# Autodesk Inventor assembly: legg_assembly
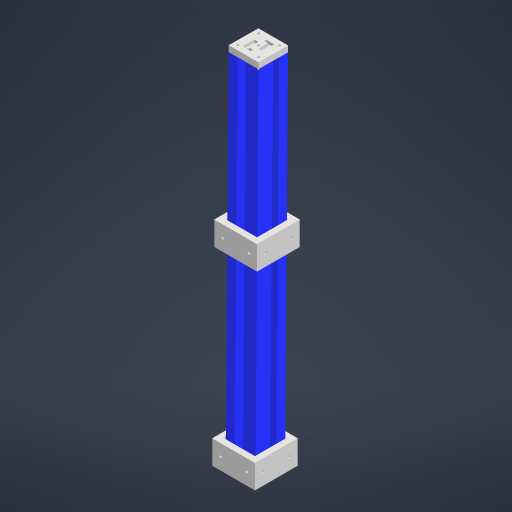
[picture p0: Inventor's stored thumbnail of the model, 512x512]
Saved by Autodesk Inventor 2024 (Build 280153000, 153)
## iProperties
Created: 2023-05-23
Part Number: legg_assembly
Document SubType Name: Assembly
Designer: aasmu
Author: aasmu
## Documents named in this file (4)
- C:\Users\aasmu\Documents\standing_desk\legg_assembly.iam
- C:\Users\aasmu\Documents\standing_desk\1_inner_leg.ipt
- C:\Users\aasmu\Documents\standing_desk\2_inner_leg_top_plate.ipt
- C:\Users\aasmu\Documents\standing_desk\inner_glide_cartrige_full_assembly.iam
## Components (4 placed, 3 different names)
1. 1_inner_leg:1 — Rigid:1, Tangent:1, Tangent:2, Rotation/Translation:1, Tangent:3
2. inner_glide_cartrige_full_assembly:1 [sub-assembly] — Rotation/Translation:1, Tangent:3
3. inner_glide_cartrige_full_assembly:2 [sub-assembly] — Tangent:1, Tangent:2
4. 2_inner_leg_top_plate:1 — Rigid:1
## Relationships (5: Tangent 3, WeldJoint 1, RelateRotateTranslate 1)
- Rigid:1 [WeldJoint]: 1_inner_leg:1 ↔ 2_inner_leg_top_plate:1
- Tangent:1: 1_inner_leg:1 ↔ inner_glide_cartrige_full_assembly:2
- Tangent:2: 1_inner_leg:1 ↔ inner_glide_cartrige_full_assembly:2
- Rotation/Translation:1 [RelateRotateTranslate] (1 mm): 1_inner_leg:1 ↔ inner_glide_cartrige_full_assembly:1
- Tangent:3: 1_inner_leg:1 ↔ inner_glide_cartrige_full_assembly:1
